# Autodesk Inventor assembly: Exam-3_Leo Berman_Assembly
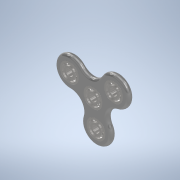
[picture p0: Inventor's stored thumbnail of the model, 180x180]
Saved by Autodesk Inventor 2022 (Build 260153000, 153)
## iProperties
Created: 2022-03-30
Part Number: Exam-3_Leo Berman_Assembly
Document SubType Name: Assembly
Designer: leogr
Author: leogr
## Documents named in this file (4)
- C:\Users\leogr\Temple University\Semester 2\Engineering Graphics\Inventor Projects\Inventor Projects\Engineering Graphics\Exam-3_Leo Berman_Assembly.iam
- C:\Users\leogr\Temple University\Semester 2\Engineering Graphics\Inventor Projects\Inventor Projects\Engineering Graphics\Exam 3_03-30-2022 Leo Berman.ipt
- C:\Users\leogr\Temple University\Semester 2\Engineering Graphics\Inventor Projects\Inventor Projects\Engineering Graphics\Exam-3_Leo Berman_Assembly\Design Accelerator\Bearing1.iam
- C:\Users\leogr\Temple University\Semester 2\Engineering Graphics\Inventor Projects\Inventor Projects\Engineering Graphics\Exam-3_Leo Berman_Assembly\Design Accelerator\Bearing2.iam
## Components (5 placed, 2 different names)
1. Exam 3_03-30-2022 Leo Berman:1 — Mate:1, Mate:2, Flush:1, Flush:2, Flush:3, Flush:4, Flush:5, Mate:5
2. Bearing:1 [sub-assembly] — Mate:1, Mate:3, Mate:4, Flush:2, Mate:5
3. Bearing:2 [sub-assembly] — Mate:2, Flush:3
4. Bearing:3 [sub-assembly] — Flush:5
5. Bearing:4 [sub-assembly] — Flush:4
## Component patterns: (3 elements, first: Bearing:2)
## Relationships (10: Mate 5, Flush 5)
- Mate:1: Exam 3_03-30-2022 Leo Berman:1 ↔ Bearing:1
- Mate:2: Exam 3_03-30-2022 Leo Berman:1 ↔ Bearing:2
- Mate:3: Bearing:1
- Mate:4: Bearing:1
- Flush:1: Exam 3_03-30-2022 Leo Berman:1
- Flush:2: Exam 3_03-30-2022 Leo Berman:1 ↔ Bearing:1
- Flush:3: Exam 3_03-30-2022 Leo Berman:1 ↔ Bearing:2
- Flush:4: Exam 3_03-30-2022 Leo Berman:1 ↔ Bearing:4
- Flush:5: Exam 3_03-30-2022 Leo Berman:1 ↔ Bearing:3
- Mate:5: Exam 3_03-30-2022 Leo Berman:1 ↔ Bearing:1
